# Autodesk Inventor assembly: cam(EX)
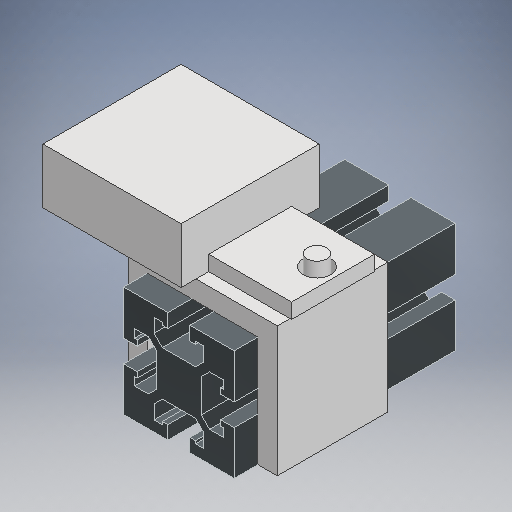
[picture p0: Inventor's stored thumbnail of the model, 512x512]
Saved by Autodesk Inventor 2025.2 (Build 292293000, 293)
## iProperties
Created: 2025-03-10
Part Number: cam(EX)
Document SubType Name: Assembly
Designer: jbhma
Author: jbhma
## Documents named in this file (4)
- C:\Users\jbhma\OneDrive\Desktop\2025_ACCA\2024 ERP42\cam(EX).iam
- C:\Users\jbhma\OneDrive\Desktop\2025_ACCA\2024 ERP42\프로파일\8.ipt
- C:\Users\jbhma\OneDrive\Desktop\2025_ACCA\2024 ERP42\camera_case_jbh.ipt
- C:\Users\jbhma\OneDrive\Desktop\2025_ACCA\2024 ERP42\camsera_case_girl.ipt
## Components (3 placed, 3 different names)
1. 8:1 — 메이트:1, 메이트:2
2. camera_case_jbh:1 — 메이트:1, 메이트:2, 각도:1, 메이트:3
3. camsera_case_girl:1 — 각도:1, 메이트:3
## Relationships (4: Mate 3, Angle 1)
- 메이트:1 [Mate]: 8:1 ↔ camera_case_jbh:1
- 메이트:2 [Mate]: 8:1 ↔ camera_case_jbh:1
- 각도:1 [Angle] (180 deg): camera_case_jbh:1 ↔ camsera_case_girl:1
- 메이트:3 [Mate]: camera_case_jbh:1 ↔ camsera_case_girl:1
